# Autodesk Inventor assembly: inner_w_hardware_mirrored
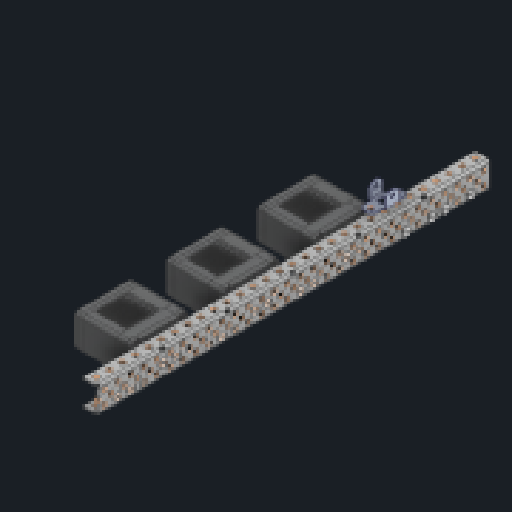
[picture p0: Inventor's stored thumbnail of the model, 512x512]
Saved by Autodesk Inventor 2025 (Build 290162000, 162)
## iProperties
Created: 2024-10-11
Part Number: inner_w_hardware_mirrored
Document SubType Name: Assembly
Designer: Averey Ku
Author: Averey Ku
## Documents named in this file (7)
- D:\vex_robotics_high_stakes\hardware\cad\bots\high_stakes_v2\chassis_v2\drivebay_mirrored\inner_w_hardware_mirrored.iam
- D:\vex_robotics_high_stakes\hardware\cad\bots\high_stakes_v2\chassis_v2\drivebay_mirrored\inner_mirrored.iam
- D:\vex_robotics_high_stakes\hardware\cad\bots\high_stakes_v2\chassis_v2\drivebay_mirrored\V5 Motor_mirrored.ipt
- D:\vex_robotics_high_stakes\hardware\cad\bots\high_stakes_v2\chassis_v2\drivebay_mirrored\NScrew Slotted Threaded .500_mirrored.ipt
- D:\vex_robotics_high_stakes\hardware\cad\bots\high_stakes_v2\chassis_v2\drivebay_mirrored\bearing_flat_w_hardware_offset_mirrored.iam
- D:\vex_robotics_high_stakes\hardware\cad\bots\high_stakes_v2\chassis_v2\drivebay_mirrored\bearing_flat_w_hardware_mirrored.iam
- D:\vex_robotics_high_stakes\hardware\cad\robpros_cad_lib\Motion\Pneumatics\Cylinder Rod Pivot.ipt
## Components (16 placed, 6 different names)
1. inner_mirrored:1 [sub-assembly] — Insert:1, Insert:2, Insert:3, Mate:2, Insert:4, Mate:3, Insert:5, Insert:6, Mate:5
2. Cylinder Rod Pivot:1 — Insert:6, Mate:5
3. V5 Motor_mirrored:1 — Insert:1, Mate:4
4. NScrew Slotted Threaded .500_mirrored:1 — Insert:2
5. NScrew Slotted Threaded .500_mirrored:2 — Insert:3, Mate:4
6. V5 Motor_mirrored:2
7. NScrew Slotted Threaded .500_mirrored:3
8. NScrew Slotted Threaded .500_mirrored:4
9. V5 Motor_mirrored:3
10. NScrew Slotted Threaded .500_mirrored:5
11. NScrew Slotted Threaded .500_mirrored:6
12. bearing_flat_w_hardware_offset_mirrored:1 [sub-assembly] — Mate:2, Insert:4
13. bearing_flat_w_hardware_offset_mirrored:2 [sub-assembly]
14. bearing_flat_w_hardware_offset_mirrored:3 [sub-assembly]
15. bearing_flat_w_hardware_mirrored:1 [sub-assembly] — Mate:3, Insert:5
16. bearing_flat_w_hardware_mirrored:2 [sub-assembly]
## Component patterns: (3 elements, first: V5 Motor_mirrored:1 + NScrew Slotted Threaded .500_mirrored:1 + NScrew Slotted Threaded .500_mirrored:2), (3 elements, first: bearing_flat_w_hardware_offset_mirrored:1), (2 elements, first: bearing_flat_w_hardware_mirrored:1)
## Relationships (10: Insert 6, Mate 4)
- Insert:1: inner_mirrored:1 ↔ V5 Motor_mirrored:1
- Insert:2: inner_mirrored:1 ↔ NScrew Slotted Threaded .500_mirrored:1
- Insert:3: inner_mirrored:1 ↔ NScrew Slotted Threaded .500_mirrored:2
- Mate:2: inner_mirrored:1 ↔ bearing_flat_w_hardware_offset_mirrored:1
- Insert:4: inner_mirrored:1 ↔ bearing_flat_w_hardware_offset_mirrored:1
- Mate:3: inner_mirrored:1 ↔ bearing_flat_w_hardware_mirrored:1
- Insert:5: inner_mirrored:1 ↔ bearing_flat_w_hardware_mirrored:1
- Mate:4: V5 Motor_mirrored:1 ↔ NScrew Slotted Threaded .500_mirrored:2
- Insert:6 (7.9375 mm): inner_mirrored:1 ↔ Cylinder Rod Pivot:1
- Mate:5: inner_mirrored:1 ↔ Cylinder Rod Pivot:1
